# Autodesk Inventor assembly: G129_Hand_Assembly
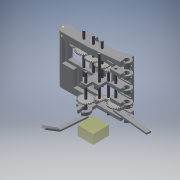
[picture p0: Inventor's stored thumbnail of the model, 180x180]
Saved by Autodesk Inventor 2017 (Build 210142000, 142)
## iProperties
Created: 2016-09-28
Part Number: G129_Hand_Assembly
Document SubType Name: Assembly
Designer: cmcdona
Author: cmcdona
## Documents named in this file (20)
- C:\Users\malik\Desktop\G129_Hand_Assembly.iam
- C:\Users\malik\Desktop\C03_Final\Hand - Frame.ipt
- C:\Users\malik\Desktop\C03_Final\Hand - Digit 4.ipt
- C:\Users\malik\Desktop\C03_Final\Hand - Digit 0-1.ipt
- C:\Users\malik\Desktop\C03_Final\Hand - Distal Bridge.ipt
- C:\Users\malik\Desktop\C03_Final\Hand - Digit 2-3.ipt
- C:\Users\malik\Desktop\C03_Final\Hand - Proximal Bridge.ipt
- C:\Users\malik\Desktop\C03_Final\Hand - Functional Workspace.ipt
- C:\Users\malik\Desktop\C03_Final\Input Motor.ipt
- C:\Users\malik\Desktop\C03_Final\Mounting bracket.ipt
- C:\Users\malik\Desktop\C03_Final\Spur Gears1.iam
- C:\Users\malik\Desktop\C03_Final\Spur Gear11.ipt
- C:\Users\malik\Desktop\C03_Final\Threaded Rod.ipt
- C:\Users\malik\Desktop\C03_Final\Spur Gears2.iam
- C:\Users\malik\Desktop\C03_Final\Spur Gear12.ipt
- C:\Users\malik\Desktop\C03_Final\Spur Gear22.ipt
- C:\Users\malik\Desktop\C03_Final\Spur Gears3.iam
- C:\Users\malik\Desktop\C03_Final\Spur Gears4.iam
- C:\Users\malik\Desktop\C03_Final\Thumb.ipt
- C:\Users\malik\Desktop\C03_Final\Finger.ipt
## Components (34 placed, 15 different names)
1. Hand - Frame:1 — Flush:1, Flush:2, Mate:1, Mate:2, Flush:3, Mate:3, Mate:16, Mate:17, Mate:18, Mate:22, Mate:23, Mate:25, Mate:27, Mate:64, Mate:79
2. Hand - Digit 4:1 — Flush:1, Flush:2, Mate:1, Mate:4, Mate:5
3. Hand - Digit 0-1:1 — Mate:2, Flush:3, Mate:3, Mate:6, Mate:19, Mate:20, Mate:21
4. Hand - Distal Bridge:1 — Mate:4, Mate:5, Mate:6, Mate:7, Mate:8, Mate:9, Mate:10, Mate:11, Mate:12, Mate:13, Mate:14, Mate:15
5. Hand - Digit 2-3:1 — Mate:7, Mate:8, Mate:9
6. Hand - Digit 2-3:2 — Mate:10, Mate:11, Mate:12
7. Hand - Digit 2-3:3 — Mate:13, Mate:14, Mate:15
8. Hand - Proximal Bridge:1 — Mate:16, Mate:17, Mate:18
9. Hand - Functional Workspace:1 — Mate:19, Mate:20, Mate:21
10. Input Motor:1 — Mate:25, Mate:26, Flush:4, Mate:27, Mate:78, Mate:79
11. Mounting bracket:1 — Mate:22, Mate:23, Flush:5, Mate:28, Flush:6, Flush:7, Mate:29, Mate:31, Mate:35, Mate:39, Mate:43, Mate:44, Mate:47, Mate:49, Mate:51, Mate:53, Flush:11, Mate:78, Mate:80
12. Spur Gears:1 [sub-assembly]
13. Spur Gear1:1 — Mate:26, Flush:4, Rotation:1
14. Threaded Rod:1 — Flush:7, Mate:29, Mate:30, Mate:32, Mate:76, Mate:77
15. Spur Gears:2 [sub-assembly]
16. Spur Gear1:2 — Mate:30, Mate:31, Mate:33, Mate:76, Rotation:1
17. Spur Gear2:1 — Mate:32, Mate:33, Mate:77, Rotation:2
18. Threaded Rod:2 — Mate:28, Flush:6, Mate:34, Mate:36, Mate:65, Mate:75
19. Threaded Rod:3 — Flush:5, Mate:38, Mate:40, Mate:47, Mate:66, Mate:74
20. Spur Gear1:3 — Mate:52, Mate:53, Mate:69, Rotation:6, Flush:14
21. Spur Gear1:4 — Mate:34, Mate:35, Mate:37, Mate:75, Rotation:2
22. Spur Gear2:2 — Flush:9, Mate:42, Mate:44, Mate:67, Rotation:4
23. Spur Gear2:3 — Mate:40, Mate:41, Mate:66, Rotation:4
24. Spur Gear2:4 — Mate:36, Mate:37, Mate:65, Rotation:3
25. Spur Gears:3 [sub-assembly] — Mate:38, Mate:39, Mate:41, Mate:74, Rotation:3
26. Threaded Rod:4 — Flush:9, Mate:42, Mate:43, Mate:48, Mate:67, Mate:71
27. Spur Gear2:5 — Mate:48, Flush:12, Flush:13, Mate:71, Rotation:5, Rotation:7
28. Spur Gears:4 [sub-assembly] — Flush:10, Mate:50, Flush:12, Mate:68, Rotation:5, Rotation:6, Flush:14
29. Spur Gear1:5 — Mate:55, Flush:13, Mate:73, Rotation:7
30. Threaded Rod:5 — Mate:51, Mate:52, Flush:11, Mate:60, Mate:61, Mate:69, Mate:70
31. Threaded Rod:6 — Mate:49, Flush:10, Mate:50, Mate:68
32. Threaded Rod:7 — Mate:55, Mate:62, Mate:63, Mate:64, Mate:72, Mate:73, Mate:80
33. Thumb:1 — Mate:60, Mate:61, Mate:70
34. Finger:1 — Mate:62, Mate:63, Mate:72
## Relationships (92: Mate 72, Flush 13, RelateRotation 7)
- Flush:1: Hand - Frame:1 ↔ Hand - Digit 4:1
- Flush:2: Hand - Frame:1 ↔ Hand - Digit 4:1
- Mate:1: Hand - Frame:1 ↔ Hand - Digit 4:1
- Mate:2: Hand - Frame:1 ↔ Hand - Digit 0-1:1
- Flush:3: Hand - Frame:1 ↔ Hand - Digit 0-1:1
- Mate:3: Hand - Frame:1 ↔ Hand - Digit 0-1:1
- Mate:4: Hand - Digit 4:1 ↔ Hand - Distal Bridge:1
- Mate:5: Hand - Digit 4:1 ↔ Hand - Distal Bridge:1
- Mate:6: Hand - Digit 0-1:1 ↔ Hand - Distal Bridge:1
- Mate:7: Hand - Distal Bridge:1 ↔ Hand - Digit 2-3:1
- Mate:8: Hand - Distal Bridge:1 ↔ Hand - Digit 2-3:1
- Mate:9: Hand - Distal Bridge:1 ↔ Hand - Digit 2-3:1
- Mate:10: Hand - Distal Bridge:1 ↔ Hand - Digit 2-3:2
- Mate:11: Hand - Distal Bridge:1 ↔ Hand - Digit 2-3:2
- Mate:12: Hand - Distal Bridge:1 ↔ Hand - Digit 2-3:2
- Mate:13: Hand - Distal Bridge:1 ↔ Hand - Digit 2-3:3
- Mate:14: Hand - Distal Bridge:1 ↔ Hand - Digit 2-3:3
- Mate:15: Hand - Distal Bridge:1 ↔ Hand - Digit 2-3:3
- Mate:16: Hand - Frame:1 ↔ Hand - Proximal Bridge:1
- Mate:17: Hand - Frame:1 ↔ Hand - Proximal Bridge:1
- Mate:18: Hand - Frame:1 ↔ Hand - Proximal Bridge:1
- Mate:19: Hand - Digit 0-1:1 ↔ Hand - Functional Workspace:1
- Mate:20 (41 mm): Hand - Digit 0-1:1 ↔ Hand - Functional Workspace:1
- Mate:21 (33 mm): Hand - Digit 0-1:1 ↔ Hand - Functional Workspace:1
- Mate:22: Hand - Frame:1 ↔ Mounting bracket:1
- Mate:23: Hand - Frame:1 ↔ Mounting bracket:1
- Mate:25: Hand - Frame:1 ↔ Input Motor:1
- Mate:26: Input Motor:1 ↔ Spur Gear1:1
- Flush:4: Input Motor:1 ↔ Spur Gear1:1
- Mate:27: Hand - Frame:1 ↔ Input Motor:1
- Flush:5 (-10 mm): Mounting bracket:1 ↔ Threaded Rod:3
- Mate:28: Mounting bracket:1 ↔ Threaded Rod:2
- Flush:6 (-10 mm): Mounting bracket:1 ↔ Threaded Rod:2
- Flush:7 (-10 mm): Mounting bracket:1 ↔ Threaded Rod:1
- Mate:29: Mounting bracket:1 ↔ Threaded Rod:1
- Mate:30: Threaded Rod:1 ↔ Spur Gear1:2
- Mate:31 (1 mm): Mounting bracket:1 ↔ Spur Gear1:2
- Mate:32: Threaded Rod:1 ↔ Spur Gear2:1
- Mate:33 (1 mm): Spur Gear1:2 ↔ Spur Gear2:1
- Mate:34: Threaded Rod:2 ↔ Spur Gear1:4
- Mate:35 (4 mm): Mounting bracket:1 ↔ Spur Gear1:4
- Mate:36: Threaded Rod:2 ↔ Spur Gear2:4
- Mate:37 (1 mm): Spur Gear1:4 ↔ Spur Gear2:4
- Mate:38: Threaded Rod:3 ↔ Spur Gears:3
- Mate:39 (7 mm): Mounting bracket:1 ↔ Spur Gears:3
- Mate:40: Threaded Rod:3 ↔ Spur Gear2:3
- Mate:41 (1 mm): Spur Gear2:3 ↔ Spur Gears:3
- Flush:9: Spur Gear2:2 ↔ Threaded Rod:4
- Mate:42: Spur Gear2:2 ↔ Threaded Rod:4
- Mate:43: Mounting bracket:1 ↔ Threaded Rod:4
- Mate:44 (10 mm): Mounting bracket:1 ↔ Spur Gear2:2
- Mate:47: Mounting bracket:1 ↔ Threaded Rod:3
- Mate:48: Threaded Rod:4 ↔ Spur Gear2:5
- Mate:49: Mounting bracket:1 ↔ Threaded Rod:6
- Flush:10: Spur Gears:4 ↔ Threaded Rod:6
- Mate:50: Spur Gears:4 ↔ Threaded Rod:6
- Mate:51: Mounting bracket:1 ↔ Threaded Rod:5
- Mate:52: Spur Gear1:3 ↔ Threaded Rod:5
- Mate:53 (22 mm): Mounting bracket:1 ↔ Spur Gear1:3
- Flush:11 (-18 mm): Mounting bracket:1 ↔ Threaded Rod:5
- Mate:55: Spur Gear1:5 ↔ Threaded Rod:7
- Mate:60: Threaded Rod:5 ↔ Thumb:1
- Mate:61 (-4 mm): Threaded Rod:5 ↔ Thumb:1
- Mate:62: Threaded Rod:7 ↔ Finger:1
- Mate:63 (-7 mm): Threaded Rod:7 ↔ Finger:1
- Flush:12: Spur Gear2:5 ↔ Spur Gears:4
- Mate:64 (10 mm): Hand - Frame:1 ↔ Threaded Rod:7
- Flush:13: Spur Gear2:5 ↔ Spur Gear1:5
- Mate:65: Threaded Rod:2 ↔ Spur Gear2:4
- Mate:66: Threaded Rod:3 ↔ Spur Gear2:3
- Mate:67: Spur Gear2:2 ↔ Threaded Rod:4
- Mate:68: Spur Gears:4 ↔ Threaded Rod:6
- Mate:69: Spur Gear1:3 ↔ Threaded Rod:5
- Mate:70: Threaded Rod:5 ↔ Thumb:1
- Mate:71: Threaded Rod:4 ↔ Spur Gear2:5
- Mate:72: Threaded Rod:7 ↔ Finger:1
- Mate:73: Spur Gear1:5 ↔ Threaded Rod:7
- Mate:74: Threaded Rod:3 ↔ Spur Gears:3
- Mate:75: Threaded Rod:2 ↔ Spur Gear1:4
- Mate:76: Threaded Rod:1 ↔ Spur Gear1:2
- Mate:77: Threaded Rod:1 ↔ Spur Gear2:1
- Rotation:1 [RelateRotation] (0.5 ul): Spur Gear1:1 ↔ Spur Gear1:2
- Rotation:2 [RelateRotation] (0.5 ul): Spur Gear2:1 ↔ Spur Gear1:4
- Rotation:3 [RelateRotation] (0.5714 ul): Spur Gear2:4 ↔ Spur Gears:3
- Rotation:4 [RelateRotation] (1 ul): Spur Gear2:2 ↔ Spur Gear2:3
- Rotation:5 [RelateRotation] (0.9231 ul): Spur Gear2:5 ↔ Spur Gears:4
- Rotation:6 [RelateRotation] (0.5417 ul): Spur Gear1:3 ↔ Spur Gears:4
- Rotation:7 [RelateRotation] (0.5 ul): Spur Gear2:5 ↔ Spur Gear1:5
- Flush:14: Spur Gear1:3 ↔ Spur Gears:4
- Mate:78: Input Motor:1 ↔ Mounting bracket:1
- Mate:79: Hand - Frame:1 ↔ Input Motor:1
- Mate:80: Mounting bracket:1 ↔ Threaded Rod:7
